# Autodesk Inventor assembly: Parameter
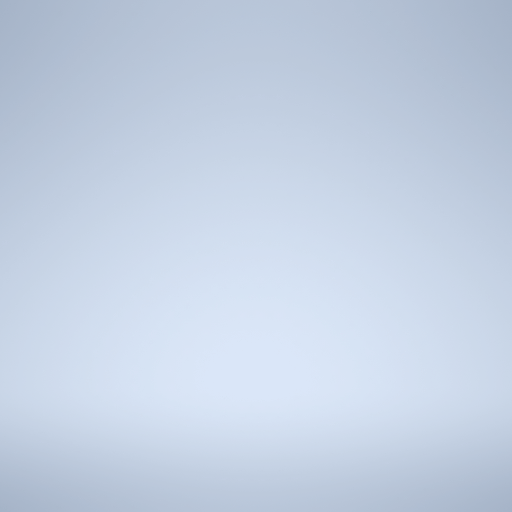
[picture p0: Inventor's stored thumbnail of the model, 512x512]
Saved by Autodesk Inventor 2025 (Build 290162010, 162A)
## iProperties
Created: 2024-11-20
Part Number: Parameter
Document SubType Name: Assembly
Designer: Admin
schrägWinkel: 1,61 grd
höheFrame: 475,000 mm
seildurchmesser: 2,000 mm
Author: Admin
## Documents named in this file (1)
- C:\Users\Admin\Documents\Inventor\Krandemonstrator\Parameter.iam
## Named parameters: schrägWinkel = 1.614505 deg, höheFrame = 475 mm, seildurchmesser = 2 mm
